# Autodesk Inventor assembly: 1561 Daughter Board Populated
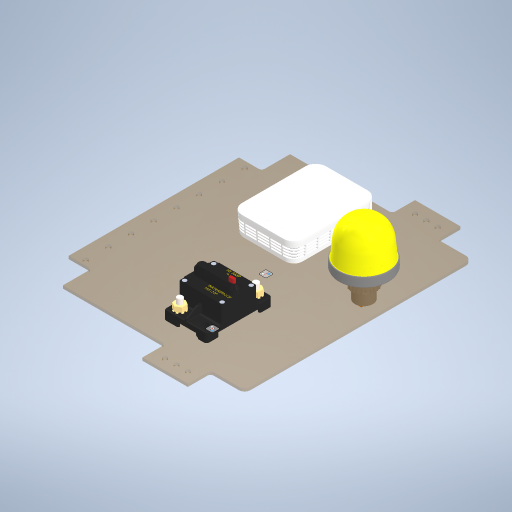
[picture p0: Inventor's stored thumbnail of the model, 512x512]
Saved by Autodesk Inventor 2023.3 (Build 273359000, 359)
## iProperties
Created: 2023-10-01
Part Number: 1561 Daughter Board Populated
Document SubType Name: Assembly
Designer: jackc
Author: jackc
## Documents named in this file (5)
- D:\.shortcut-targets-by-id\104lhnwPhYvankLacu8RGROV89Bx_24Mg\1939\2_Design\2023-2024\Parts\Electrical Panels\1561 Daughter Board Populated.iam
- D:\.shortcut-targets-by-id\104lhnwPhYvankLacu8RGROV89Bx_24Mg\1939\2_Design\2023-2024\Parts\Electrical Panels\1561 Daughter Board.ipt
- D:\.shortcut-targets-by-id\104lhnwPhYvankLacu8RGROV89Bx_24Mg\1939\2_Design\2023-2024\Parts\Electronics\am-3583 Generic RSL.ipt
- D:\.shortcut-targets-by-id\104lhnwPhYvankLacu8RGROV89Bx_24Mg\1939\2_Design\2023-2024\Parts\Electronics\OM5P-AC_Radio.ipt
- D:\.shortcut-targets-by-id\104lhnwPhYvankLacu8RGROV89Bx_24Mg\1939\2_Design\2023-2024\Parts\Electronics\am-0282 120a Circuit Breaker.ipt
## Components (4 placed, 4 different names)
1. 1561 Daughter Board:1 — Mate:1, Mate:2, Mate:3, Mate:5, Mate:6, Mate:7, Mate:8, Mate:9
2. am-3583 Generic RSL:1 — Mate:6, Mate:7
3. OM5P-AC_Radio:1 — Mate:1, Mate:2, Mate:3
4. am-0282 120a Circuit Breaker:1 — Mate:5, Mate:8, Mate:9
## Relationships (8: Mate 8)
- Mate:1: 1561 Daughter Board:1 ↔ OM5P-AC_Radio:1
- Mate:2: 1561 Daughter Board:1 ↔ OM5P-AC_Radio:1
- Mate:3: 1561 Daughter Board:1 ↔ OM5P-AC_Radio:1
- Mate:5: 1561 Daughter Board:1 ↔ am-0282 120a Circuit Breaker:1
- Mate:6: 1561 Daughter Board:1 ↔ am-3583 Generic RSL:1
- Mate:7: 1561 Daughter Board:1 ↔ am-3583 Generic RSL:1
- Mate:8: 1561 Daughter Board:1 ↔ am-0282 120a Circuit Breaker:1
- Mate:9: 1561 Daughter Board:1 ↔ am-0282 120a Circuit Breaker:1
